# Autodesk Inventor assembly: Revised Unit
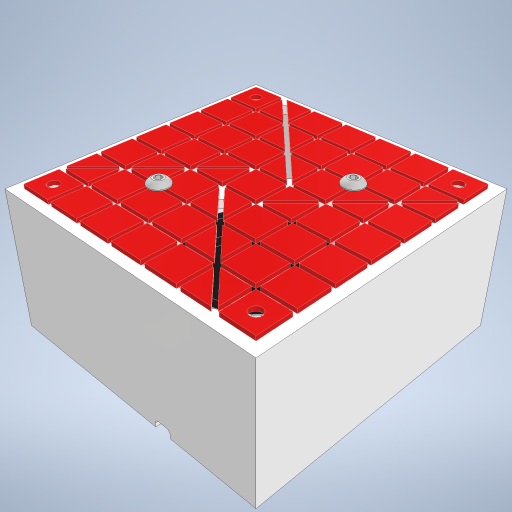
[picture p0: Inventor's stored thumbnail of the model, 512x512]
Saved by Autodesk Inventor 2024 (Build 280153000, 153)
## iProperties
Created: 2023-04-24
Part Number: Revised Unit
Document SubType Name: Assembly
Designer: byrne
Author: byrne
## Documents named in this file (12)
- C:\Users\byrne\OneDrive\Documents\Inventor\RAI\Revised Unit.iam
- C:\Users\byrne\OneDrive\Documents\Inventor\RAI\Revised Solid Unit.ipt
- C:\Users\byrne\OneDrive\Documents\Inventor\RAI\Pololu#1053 v4.ipt
- C:\Users\byrne\OneDrive\Documents\Inventor\RAI\Dual Servo Attachment.ipt
- C:\Users\byrne\OneDrive\Documents\Inventor\RAI\Rotating Disc.ipt
- C:\Users\byrne\OneDrive\Documents\Inventor\RAI\Linear Arm.ipt
- C:\Users\byrne\OneDrive\Documents\Inventor\RAI\Spacer.ipt
- C:\Users\byrne\OneDrive\Documents\Inventor\RAI\90631A009_Low-Strength Steel Nylon-Insert Locknut\90631A009_Low-Strength Steel Nylon-Insert Locknut.ipt
- C:\Users\byrne\OneDrive\Documents\Inventor\RAI\93365A140_Tapered Heat-Set Inserts for Plastic\93365A140_Tapered Heat-Set Inserts for Plastic.ipt
- C:\Users\byrne\OneDrive\Documents\Inventor\RAI\98164A134_316 Stainless Steel Button Head Hex Drive Screw\98164A134_316 Stainless Steel Button Head Hex Drive Screw.ipt
- C:\Users\byrne\OneDrive\Documents\Inventor\RAI\98164A135_316 Stainless Steel Button Head Hex Drive Screw\98164A135_316 Stainless Steel Button Head Hex Drive Screw.ipt
- C:\Users\byrne\OneDrive\Documents\Inventor\RAI\Flasher.ipt
## Components (21 placed, 11 different names)
1. Revised Solid Unit:1 — Mate:1, Mate:2, Angle:1, Mate:3, Mate:4, Mate:5, Angle:2, Mate:6
2. Pololu#1053 v4:1 — Mate:1, Mate:2, Angle:1, Insert:1
3. Dual Servo Attachment:1 — Insert:1, Insert:2, Insert:3
4. Rotating Disc:1 — Insert:2, Insert:3, Insert:4, Insert:5, Insert:16, Insert:18
5. Linear Arm:1 — Insert:4, Mate:4, Insert:7, Insert:12
6. Linear Arm:2 — Insert:5, Mate:3, Insert:6, Insert:17
7. Spacer:1 — Insert:6, Insert:9, Insert:11, Insert:20
8. Spacer:2 — Insert:7, Insert:8, Insert:10, Insert:19
9. 90631A009_Low-Strength Steel Nylon-Insert Locknut:1 — Insert:16
10. 93365A140_Tapered Heat-Set Inserts for Plastic:1 — Insert:8
11. 98164A134_316 Stainless Steel Button Head Hex Drive Screw:1 — Insert:12
12. 98164A135_316 Stainless Steel Button Head Hex Drive Screw:1 — Insert:20
13. 93365A140_Tapered Heat-Set Inserts for Plastic:2 — Insert:9
14. 93365A140_Tapered Heat-Set Inserts for Plastic:3 — Insert:11
15. 93365A140_Tapered Heat-Set Inserts for Plastic:4 — Insert:10
16. 98164A135_316 Stainless Steel Button Head Hex Drive Screw:3
17. 98164A134_316 Stainless Steel Button Head Hex Drive Screw:3 — Insert:17
18. 98164A135_316 Stainless Steel Button Head Hex Drive Screw:2
19. 90631A009_Low-Strength Steel Nylon-Insert Locknut:2 — Insert:18
20. Flasher:1 — Mate:5, Angle:2, Mate:6
21. 98164A135_316 Stainless Steel Button Head Hex Drive Screw:4 — Insert:19
## Relationships (27: Insert 19, Mate 6, Angle 2)
- Mate:1: Revised Solid Unit:1 ↔ Pololu#1053 v4:1
- Mate:2: Revised Solid Unit:1 ↔ Pololu#1053 v4:1
- Angle:1 (0 deg): Revised Solid Unit:1 ↔ Pololu#1053 v4:1
- Insert:1: Pololu#1053 v4:1 ↔ Dual Servo Attachment:1
- Insert:2: Dual Servo Attachment:1 ↔ Rotating Disc:1
- Insert:3: Dual Servo Attachment:1 ↔ Rotating Disc:1
- Insert:4: Rotating Disc:1 ↔ Linear Arm:1
- Insert:5: Rotating Disc:1 ↔ Linear Arm:2
- Mate:3: Revised Solid Unit:1 ↔ Linear Arm:2
- Mate:4: Revised Solid Unit:1 ↔ Linear Arm:1
- Insert:6: Linear Arm:2 ↔ Spacer:1
- Insert:7: Linear Arm:1 ↔ Spacer:2
- Insert:8: Spacer:2 ↔ 93365A140_Tapered Heat-Set Inserts for Plastic:1
- Insert:9: Spacer:1 ↔ 93365A140_Tapered Heat-Set Inserts for Plastic:2
- Insert:10: Spacer:2 ↔ 93365A140_Tapered Heat-Set Inserts for Plastic:4
- Insert:11: Spacer:1 ↔ 93365A140_Tapered Heat-Set Inserts for Plastic:3
- Insert:12: Linear Arm:1 ↔ 98164A134_316 Stainless Steel Button Head Hex Drive Screw:1
- [Insert]: Linear Arm:1 ↔ 98164A135_316 Stainless Steel Button Head Hex Drive Screw:2
- [Insert]: Linear Arm:2 ↔ 98164A135_316 Stainless Steel Button Head Hex Drive Screw:3
- Insert:16: Rotating Disc:1 ↔ 90631A009_Low-Strength Steel Nylon-Insert Locknut:1
- Insert:17: Linear Arm:2 ↔ 98164A134_316 Stainless Steel Button Head Hex Drive Screw:3
- Insert:18: Rotating Disc:1 ↔ 90631A009_Low-Strength Steel Nylon-Insert Locknut:2
- Mate:5: Revised Solid Unit:1 ↔ Flasher:1
- Angle:2 (0 deg): Revised Solid Unit:1 ↔ Flasher:1
- Mate:6: Revised Solid Unit:1 ↔ Flasher:1
- Insert:19 (4.9784 mm): Spacer:2 ↔ 98164A135_316 Stainless Steel Button Head Hex Drive Screw:4
- Insert:20 (4.9784 mm): Spacer:1 ↔ 98164A135_316 Stainless Steel Button Head Hex Drive Screw:1
